# Autodesk Inventor assembly: Assembly1
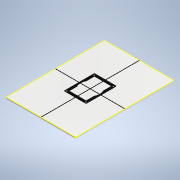
[picture p0: Inventor's stored thumbnail of the model, 180x180]
Saved by Autodesk Inventor 2020.3 (Build 243373000, 373)
## iProperties
Created: 2020-08-18
Part Number: Assembly1
Document SubType Name: Assembly
Designer: mifer
Author: mifer
## Documents named in this file (3)
- C:\Users\mifer\Desktop\PFG_USAL\Ficheros Inventor Miguel\Assembly1.iam
- C:\Users\mifer\Desktop\PFG_USAL\Ficheros Inventor Miguel\Cama.ipt
- C:\Users\mifer\Desktop\PFG_USAL\Ficheros Inventor Miguel\AdaptadorPlacaImpresión.ipt
## Components (2 placed, 2 different names)
1. Cama:1 — Mate:2
2. AdaptadorPlacaImpresión:2 — Mate:2
## Relationships (1: Mate 1)
- Mate:2: Cama:1 ↔ AdaptadorPlacaImpresión:2
